# Autodesk Inventor assembly: base_wall_added_left
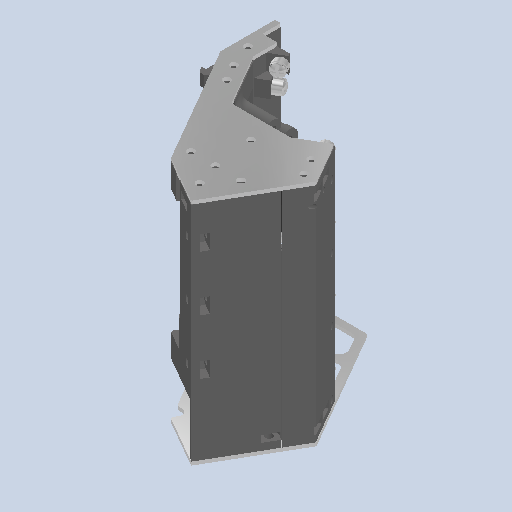
[picture p0: Inventor's stored thumbnail of the model, 512x512]
Saved by Autodesk Inventor 2024.1 (Build 281209000, 209)
## iProperties
Created: 2025-01-18
Part Number: base_wall_added_left
Document SubType Name: Assembly
Designer: hibik
Author: hibik
## Documents named in this file (3)
- C:\Users\hibik\Documents\Robomech\RESCUE\ORCA\hard\fork\left\base_wall_added_left.iam
- C:\Users\hibik\Documents\Robomech\RESCUE\ORCA\hard\fork\left\base_left.iam
- C:\Users\hibik\Documents\Robomech\RESCUE\ORCA\hard\fork\left\base_backwall_setter_upper_left.ipt
## Components (2 placed, 2 different names)
1. base_left:1 [sub-assembly] — メイト:1, フラッシュ:2, フラッシュ:1
2. base_backwall_setter_upper_left:1 — メイト:1, フラッシュ:2, フラッシュ:1
## Relationships (3: Flush 2, Mate 1)
- メイト:1 [Mate]: base_left:1 ↔ base_backwall_setter_upper_left:1
- フラッシュ:2 [Flush]: base_left:1 ↔ base_backwall_setter_upper_left:1
- フラッシュ:1 [Flush]: base_left:1 ↔ base_backwall_setter_upper_left:1
